# Autodesk Inventor assembly: caliber_truck
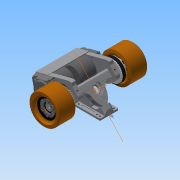
[picture p0: Inventor's stored thumbnail of the model, 180x180]
Saved by Autodesk Inventor 2015 (Build 190159000, 159)
## iProperties
Created: 2014-02-23
Part Number: caliber_truck
Document SubType Name: Assembly
Designer: Brent Yi
Author: Brent Yi
## Documents named in this file (16)
- C:\Users\brent\Documents\electric-longboard\brent\truck.iam
- C:\Users\brent\Documents\electric-longboard\brent\baseplate.ipt
- C:\Users\brent\Documents\electric-longboard\brent\hanger.ipt
- C:\Users\brent\Documents\electric-longboard\brent\mount_alt.ipt
- C:\Users\brent\Documents\electric-longboard\brent\wheel90mmwithbearing.iam
- C:\Users\brent\Documents\electric-longboard\brent\6354motor.ipt
- C:\Users\brent\Documents\electric-longboard\brent\Imported Components\15t_pulley\15t_pulley.ipt
- C:\Users\brent\Documents\electric-longboard\brent\motorguard.ipt
- C:\Users\brent\Documents\electric-longboard\brent\pulleyprotector.ipt
- C:\Users\brent\Documents\electric-longboard\brent\belt.ipt
- C:\Users\brent\Documents\electric-longboard\brent\wheel90mmwithbearing_MIR.iam
- C:\Users\brent\Documents\electric-longboard\brent\mount_alt_MIR.ipt
- C:\Users\brent\Documents\electric-longboard\brent\6354motor_MIR.ipt
- C:\Users\brent\Documents\electric-longboard\brent\Imported Components\15t_pulley\15t_pulley_MIR.ipt
- C:\Users\brent\Documents\electric-longboard\brent\pulleyprotector_MIR.ipt
- C:\Users\brent\Documents\electric-longboard\brent\belt_MIR1.ipt
## Components (16 placed, 15 different names)
1. baseplate:1 — Mate:1, Mate:2, Mate:17, Mate:30, Mate:31, Mate:35
2. hanger:1 — Mate:1, Mate:2, Mate:7, Mate:9, Mate:16, Flush:1, Mate:25, Mate:28, Mate:32, Mate:33, Mate:46, Mate:52, Angle:1, Mate:62, Mate:63, Mate:64
3. wheel90mmwithbearing:1 [sub-assembly] — Mate:7, Mate:25
4. wheel90mmwithbearing:2 [sub-assembly] — Mate:9, Mate:28
5. mount_alt:1 — Flush:1, Mate:21, Mate:32, Mate:33, Mate:34, Mate:41, Mate:42, Flush:3, Mate:49, Mate:50, Mate:51
6. 6354motor:1 — Mate:21, Mate:23, Mate:26, Mate:34, Mate:47
7. 15t_pulley:1 — Mate:23, Mate:26, Mate:48
8. motorguard:1 — Mate:41, Mate:42, Flush:3
9. pulleyprotector:1 — Mate:49, Mate:50, Mate:51
10. belt:1 — Mate:46, Mate:47, Mate:48
11. wheel90mmwithbearing_MIR:1 [sub-assembly] — Mate:62
12. mount_alt_MIR:1 — Mate:53, Mate:54, Mate:57, Mate:63, Mate:64, Mate:65, Mate:66
13. 6354motor_MIR:1 — Mate:53, Mate:54, Mate:55, Mate:56
14. 15t_pulley_MIR:1 — Mate:55, Mate:56
15. pulleyprotector_MIR:1 — Mate:57, Mate:65, Mate:66
16. belt_MIR1:1
## Relationships (39: Mate 36, Flush 2, Angle 1)
- Mate:1: baseplate:1 ↔ hanger:1
- Mate:2: baseplate:1 ↔ hanger:1
- Mate:7: hanger:1 ↔ wheel90mmwithbearing:1
- Mate:9: hanger:1 ↔ wheel90mmwithbearing:2
- Mate:16: hanger:1
- Mate:17: baseplate:1
- Flush:1 (-28.575 mm): hanger:1 ↔ mount_alt:1
- Mate:21: mount_alt:1 ↔ 6354motor:1
- Mate:23: 6354motor:1 ↔ 15t_pulley:1
- Mate:25 (1.27 mm): hanger:1 ↔ wheel90mmwithbearing:1
- Mate:26 (5.08 mm): 6354motor:1 ↔ 15t_pulley:1
- Mate:28 (1.27 mm): hanger:1 ↔ wheel90mmwithbearing:2
- Mate:30: baseplate:1
- Mate:31: baseplate:1
- Mate:32: hanger:1 ↔ mount_alt:1
- Mate:33: hanger:1 ↔ mount_alt:1
- Mate:34: mount_alt:1 ↔ 6354motor:1
- Mate:35: baseplate:1
- Mate:41: mount_alt:1 ↔ motorguard:1
- Mate:42: mount_alt:1 ↔ motorguard:1
- Flush:3: mount_alt:1 ↔ motorguard:1
- Mate:46: hanger:1 ↔ belt:1
- Mate:47: 6354motor:1 ↔ belt:1
- Mate:48 (-8.89 mm): 15t_pulley:1 ↔ belt:1
- Mate:49: mount_alt:1 ↔ pulleyprotector:1
- Mate:50: mount_alt:1 ↔ pulleyprotector:1
- Mate:51: mount_alt:1 ↔ pulleyprotector:1
- Mate:52: hanger:1
- Angle:1 (0 deg): hanger:1
- Mate:53: mount_alt_MIR:1 ↔ 6354motor_MIR:1
- Mate:54: mount_alt_MIR:1 ↔ 6354motor_MIR:1
- Mate:55 (5.08 mm): 6354motor_MIR:1 ↔ 15t_pulley_MIR:1
- Mate:56: 6354motor_MIR:1 ↔ 15t_pulley_MIR:1
- Mate:57: mount_alt_MIR:1 ↔ pulleyprotector_MIR:1
- Mate:62: hanger:1 ↔ wheel90mmwithbearing_MIR:1
- Mate:63: hanger:1 ↔ mount_alt_MIR:1
- Mate:64: hanger:1 ↔ mount_alt_MIR:1
- Mate:65: mount_alt_MIR:1 ↔ pulleyprotector_MIR:1
- Mate:66: mount_alt_MIR:1 ↔ pulleyprotector_MIR:1
